# Autodesk Inventor assembly: Shoulder base
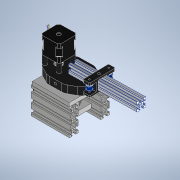
[picture p0: Inventor's stored thumbnail of the model, 180x180]
Saved by Autodesk Inventor 2022 (Build 260153000, 153)
## iProperties
Created: 2022-03-02
Part Number: Shoulder base
Document SubType Name: Assembly
Designer: JK
Author: JK
## Documents named in this file (19)
- C:\Users\JK\Documents\Inventor\ScaraNema\SCARA-3DP\Parts\Shoulder\Shoulder base.iam
- C:\Users\JK\Documents\Inventor\ScaraNema\SCARA-3DP\Parts\Shoulder\Needle roller bearing\5909K79_1 mm Thick Washer for 45 mm Shaft Diameter Needle-Roller Thrust Bearing.ipt
- C:\Users\JK\Documents\Inventor\ScaraNema\SCARA-3DP\Parts\Shoulder\Needle roller bearing\5909K19_Needle-Roller Thrust Bearing.ipt
- C:\Users\JK\Documents\Inventor\ScaraNema\SCARA-3DP\Parts\Shoulder\Platform.ipt
- C:\Users\JK\Documents\Inventor\ScaraNema\SCARA-3DP\Parts\Shoulder\Motor spacer.ipt
- C:\Users\JK\Documents\Inventor\ScaraNema\SCARA-3DP\Parts\Shoulder\MOTOR.ipt
- C:\Users\JK\Documents\Inventor\ScaraNema\SCARA-3DP\Parts\Shoulder\M3x35.ipt
- C:\Users\JK\Documents\Inventor\ScaraNema\SCARA-3DP\Parts\Shoulder\GT2 16 Pulley.ipt
- C:\Users\JK\Documents\Inventor\ScaraNema\SCARA-3DP\Parts\V-Slot 20x20\V-Slot 20x20x150.ipt
- C:\Users\JK\Documents\Inventor\ScaraNema\SCARA-3DP\Parts\V-Slot 20x20.ipt
- C:\Users\JK\Documents\Inventor\ScaraNema\SCARA-3DP\Parts\Shoulder\Belt tensor.ipt
- C:\Users\JK\Documents\Inventor\ScaraNema\SCARA-3DP\Parts\Shoulder\Idle pulley 16\GT2-16 Idle pulley.iam
- C:\Users\JK\Documents\Inventor\ScaraNema\SCARA-3DP\Parts\Shoulder\8x80 mm axis.ipt
- C:\Users\JK\Documents\Inventor\ScaraNema\SCARA-3DP\Parts\Elbow\GT260T.ipt
- C:\Users\JK\Documents\Inventor\ScaraNema\SCARA-3DP\Parts\Shoulder\KFL08 Bearing.ipt
- C:\Users\JK\Documents\Inventor\ScaraNema\SCARA-3DP\Parts\Shoulder\MOTOR_LONG.ipt
- C:\Users\JK\Documents\Inventor\ScaraNema\SCARA-3DP\Parts\Shoulder\Shoulderbasetop.ipt
- C:\Users\JK\Documents\Inventor\ScaraNema\SCARA-3DP\Parts\Shoulder\20x60x85.ipt
- C:\Users\JK\Documents\Inventor\ScaraNema\SCARA-3DP\Parts\Shoulder\Shoulderbottom.ipt
## Components (28 placed, 17 different names)
1. 5909K79_1 mm Thick Washer for 45 mm Shaft Diameter Needle-Roller Thrust Bearing:1 — Tangente:1, Coincidencia:45, Coincidencia:51
2. 5909K19_Needle-Roller Thrust Bearing:1 — Tangente:1, Tangente:2, Coincidencia:45, Coincidencia:46
3. 5909K79_1 mm Thick Washer for 45 mm Shaft Diameter Needle-Roller Thrust Bearing:2 — Tangente:2, Coincidencia:23, Coincidencia:44
4. Platform:1 — Coincidencia:23, Coincidencia:25, Coincidencia:26, Coincidencia:30, Nivelación:7, Ángulo:2, Coincidencia:32, Coincidencia:33, Nivelación:8, Coincidencia:40, Nivelación:11, Coincidencia:44
5. MOTOR:1 — Coincidencia:28, Coincidencia:31, Ángulo:2, Coincidencia:32, Coincidencia:34
6. GT2 16 Pulley:1 — Coincidencia:31, Nivelación:7
7. V-Slot 20x20x150:1 — Coincidencia:33, Nivelación:8, Coincidencia:34, Coincidencia:35, Coincidencia:36, Nivelación:9
8. Belt tensor:1 — Coincidencia:35, Coincidencia:36, Nivelación:9, Coincidencia:37, Coincidencia:38, Coincidencia:39
9. GT2-16 Idle pulley:1 [sub-assembly] — Coincidencia:37, Nivelación:10, Coincidencia:39
10. GT2-16 Idle pulley:2 [sub-assembly] — Coincidencia:38, Nivelación:10
11. 8x80 mm axis:1 — Coincidencia:40, Nivelación:11, Coincidencia:41, Coincidencia:42, Coincidencia:43, Coincidencia:46, Coincidencia:50
12. GT260T:1 — Coincidencia:41, Nivelación:12, Coincidencia:54, Coincidencia:55, Coincidencia:60
13. KFL08 Bearing:1 — Coincidencia:42, Coincidencia:55, Coincidencia:59, Coincidencia:61
14. KFL08 Bearing:2 — Coincidencia:43, Coincidencia:52, Coincidencia:53, Coincidencia:54
15. MOTOR_LONG:1 — Coincidencia:47, Coincidencia:48, Ángulo:4
16. GT2 16 Pulley:2 — Coincidencia:47, Nivelación:12, Coincidencia:48
17. Shoulderbasetop:1 — Coincidencia:50, Coincidencia:51, Coincidencia:52, Coincidencia:53, Ángulo:3, Ángulo:4, Coincidencia:57, Coincidencia:58, Nivelación:13, Nivelación:14, Nivelación:16
18. 20x60x85:1 — Coincidencia:57, Nivelación:14, Nivelación:15
19. 20x60x85:2 — Coincidencia:58, Nivelación:13, Nivelación:15, Nivelación:16
20. Shoulderbottom:1 — Coincidencia:59, Coincidencia:60, Coincidencia:61
21. M3x35:1 — Coincidencia:29, Coincidencia:30
22. Motor spacer:1 — Coincidencia:25, Coincidencia:26, Coincidencia:28, Coincidencia:29
23. M3x35:2
24. Motor spacer:2
25. M3x35:3
26. Motor spacer:3
27. M3x35:4
28. Motor spacer:4
## Component patterns: (4 elements, first: M3x35:1 + Motor spacer:1)
## Relationships (50: Mate 35, Flush 10, Angle 3, Tangent 2)
- Tangente:1: 5909K79_1 mm Thick Washer for 45 mm Shaft Diameter Needle-Roller Thrust Bearing:1 ↔ 5909K19_Needle-Roller Thrust Bearing:1
- Tangente:2: 5909K19_Needle-Roller Thrust Bearing:1 ↔ 5909K79_1 mm Thick Washer for 45 mm Shaft Diameter Needle-Roller Thrust Bearing:2
- Coincidencia:23 [Mate]: 5909K79_1 mm Thick Washer for 45 mm Shaft Diameter Needle-Roller Thrust Bearing:2 ↔ Platform:1
- Coincidencia:25 [Mate]: Platform:1 ↔ Motor spacer:1
- Coincidencia:26 [Mate]: Platform:1 ↔ Motor spacer:1
- Coincidencia:28 [Mate]: MOTOR:1 ↔ Motor spacer:1
- Coincidencia:29 [Mate]: M3x35:1 ↔ Motor spacer:1
- Coincidencia:30 [Mate]: Platform:1 ↔ M3x35:1
- Coincidencia:31 [Mate]: MOTOR:1 ↔ GT2 16 Pulley:1
- Nivelación:7 [Flush] (-6.25 mm): Platform:1 ↔ GT2 16 Pulley:1
- Ángulo:2 [Angle] (90 deg): Platform:1 ↔ MOTOR:1
- Coincidencia:32 [Mate]: Platform:1 ↔ MOTOR:1
- Coincidencia:33 [Mate]: Platform:1 ↔ V-Slot 20x20x150:1
- Nivelación:8 [Flush] (-25 mm): Platform:1 ↔ V-Slot 20x20x150:1
- Coincidencia:34 [Mate] (10 mm): MOTOR:1 ↔ V-Slot 20x20x150:1
- Coincidencia:35 [Mate] (0.15 mm): V-Slot 20x20x150:1 ↔ Belt tensor:1
- Coincidencia:36 [Mate] (0.15 mm): V-Slot 20x20x150:1 ↔ Belt tensor:1
- Nivelación:9 [Flush] (-50 mm): V-Slot 20x20x150:1 ↔ Belt tensor:1
- Coincidencia:37 [Mate]: Belt tensor:1 ↔ GT2-16 Idle pulley:1
- Coincidencia:38 [Mate]: Belt tensor:1 ↔ GT2-16 Idle pulley:2
- Nivelación:10 [Flush]: GT2-16 Idle pulley:1 ↔ GT2-16 Idle pulley:2
- Coincidencia:39 [Mate] (4 mm): Belt tensor:1 ↔ GT2-16 Idle pulley:1
- Coincidencia:40 [Mate]: Platform:1 ↔ 8x80 mm axis:1
- Nivelación:11 [Flush]: Platform:1 ↔ 8x80 mm axis:1
- Coincidencia:41 [Mate]: 8x80 mm axis:1 ↔ GT260T:1
- Coincidencia:42 [Mate]: 8x80 mm axis:1 ↔ KFL08 Bearing:1
- Coincidencia:43 [Mate]: 8x80 mm axis:1 ↔ KFL08 Bearing:2
- Coincidencia:44 [Mate]: 5909K79_1 mm Thick Washer for 45 mm Shaft Diameter Needle-Roller Thrust Bearing:2 ↔ Platform:1
- Coincidencia:45 [Mate]: 5909K79_1 mm Thick Washer for 45 mm Shaft Diameter Needle-Roller Thrust Bearing:1 ↔ 5909K19_Needle-Roller Thrust Bearing:1
- Coincidencia:46 [Mate]: 5909K19_Needle-Roller Thrust Bearing:1 ↔ 8x80 mm axis:1
- Coincidencia:47 [Mate]: MOTOR_LONG:1 ↔ GT2 16 Pulley:2
- Nivelación:12 [Flush]: GT260T:1 ↔ GT2 16 Pulley:2
- Coincidencia:48 [Mate] (2 mm): MOTOR_LONG:1 ↔ GT2 16 Pulley:2
- Coincidencia:50 [Mate]: 8x80 mm axis:1 ↔ Shoulderbasetop:1
- Coincidencia:51 [Mate]: 5909K79_1 mm Thick Washer for 45 mm Shaft Diameter Needle-Roller Thrust Bearing:1 ↔ Shoulderbasetop:1
- Coincidencia:52 [Mate]: KFL08 Bearing:2 ↔ Shoulderbasetop:1
- Coincidencia:53 [Mate]: KFL08 Bearing:2 ↔ Shoulderbasetop:1
- Coincidencia:54 [Mate]: GT260T:1 ↔ KFL08 Bearing:2
- Coincidencia:55 [Mate]: GT260T:1 ↔ KFL08 Bearing:1
- Ángulo:3 [Angle] (0 deg): Shoulderbasetop:1
- Ángulo:4 [Angle] (0 deg): MOTOR_LONG:1 ↔ Shoulderbasetop:1
- Coincidencia:57 [Mate]: Shoulderbasetop:1 ↔ 20x60x85:1
- Coincidencia:58 [Mate]: Shoulderbasetop:1 ↔ 20x60x85:2
- Nivelación:13 [Flush]: Shoulderbasetop:1 ↔ 20x60x85:2
- Nivelación:14 [Flush]: Shoulderbasetop:1 ↔ 20x60x85:1
- Nivelación:15 [Flush]: 20x60x85:1 ↔ 20x60x85:2
- Nivelación:16 [Flush]: Shoulderbasetop:1 ↔ 20x60x85:2
- Coincidencia:59 [Mate]: KFL08 Bearing:1 ↔ Shoulderbottom:1
- Coincidencia:60 [Mate]: GT260T:1 ↔ Shoulderbottom:1
- Coincidencia:61 [Mate]: KFL08 Bearing:1 ↔ Shoulderbottom:1
